# Autodesk Inventor assembly: Rexroth_Schraube_Mutter_modifiziert
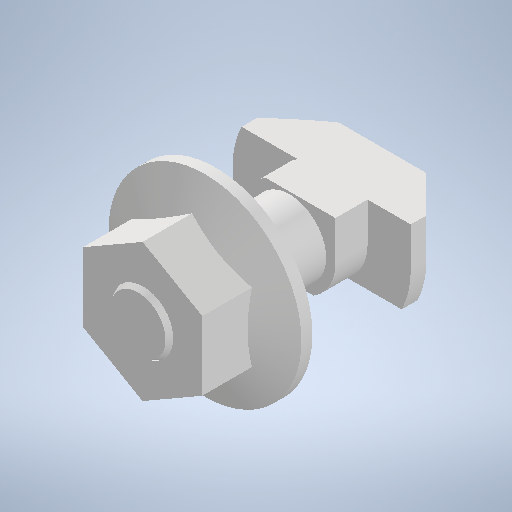
[picture p0: Inventor's stored thumbnail of the model, 512x512]
Saved by Autodesk Inventor 2025.2 (Build 292293000, 293)
## iProperties
Company: CADClick - www.CADClick.com
Created: 2025-06-16
Part Number: Rexroth_Schraube_Mutter_modifiziert
Description: STEP AP203
Document SubType Name: Assembly
Designer: Erik
Authority: unknown authorization
Preprocessor: Spatial InterOp 3D
Title: cctmp_1EE9FB96-FD97-4067-836D-2D108D3755D5_2025_06_16_13_09_51_0454_12732..stp
Author: KiM GmbH
## Documents named in this file (3)
- D:\Useless_Box\CAD-Paspa\Useless Box\Eigene Bauteile\JH_Greifer_Unterlegscheibe\Eigene Bauteile\Rexroth_Schraube_Mutter_modifiziert.iam
- D:\Useless_Box\CAD-Paspa\Useless Box\Kaufteile\Winkel_Rexroth_40x40\1.ipt
- D:\Useless_Box\CAD-Paspa\Useless Box\Kaufteile\Winkel_Rexroth_40x40\2.ipt
## Components (2 placed, 2 different names)
1. 1 — Fluchtend:1, Fluchtend:2, Fluchtend:3, Fluchtend:7
2. 2 — Fluchtend:4, Fluchtend:5, Fluchtend:6, Fluchtend:8
## Relationships (8: Flush 8)
- Fluchtend:1 [Flush]: 1
- Fluchtend:2 [Flush]: 1
- Fluchtend:3 [Flush]: 1
- Fluchtend:4 [Flush]: 2
- Fluchtend:5 [Flush]: 2
- Fluchtend:6 [Flush]: 2
- Fluchtend:7 [Flush] (-6.5 mm): 1
- Fluchtend:8 [Flush] (-4.25 mm): 2
